# Autodesk Inventor assembly: sled
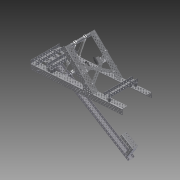
[picture p0: Inventor's stored thumbnail of the model, 180x180]
Saved by Autodesk Inventor 2014 SP1 (Build 180222100, 222)
## iProperties
Created: 2014-02-27
Part Number: sled
Document SubType Name: Assembly
Designer: Ryan
Author: Ryan
## Documents named in this file (28)
- C:\Users\Ryan\Desktop\sw\toss up 4th robot\intake\sled.iam
- C:\Users\Ryan\Desktop\sw\lib\Aperture VEX CAD Library\Metal\L Bar\2 x 35.ipt
- C:\Users\Ryan\Desktop\sw\lib\Aperture VEX CAD Library\Standoffs\BEAM-0500.ipt
- C:\Users\Ryan\Desktop\sw\lib\Aperture VEX CAD Library\Spacers\SPACER-0500-0125.ipt
- C:\Users\Ryan\Desktop\sw\lib\Aperture VEX CAD Library\Metal\C Channel\2 x 11.ipt
- C:\Users\Ryan\Desktop\sw\lib\Aperture VEX CAD Library\Metal\Plate\2 x 7.ipt
- C:\Users\Ryan\Desktop\sw\lib\Aperture VEX CAD Library\Metal\vex hinge\hinge.iam
- C:\Users\Ryan\Desktop\sw\lib\Aperture VEX CAD Library\Metal\C Channel\2 x 35.ipt
- C:\Users\Ryan\Desktop\sw\lib\Aperture VEX CAD Library\Spacers\SPACER-0500-0500.ipt
- C:\Users\Ryan\Desktop\sw\lib\Aperture VEX CAD Library\Metal\L Bar\2 x 14.ipt
- C:\Users\Ryan\Desktop\sw\lib\Aperture VEX CAD Library\Hardware\8-32\8-32_.375.ipt
- C:\Users\Ryan\Desktop\sw\lib\Aperture VEX CAD Library\Metal\Custom 1 bar\4 holes.ipt
- C:\Users\Ryan\Desktop\sw\lib\Aperture VEX CAD Library\Bearing Blocks\Bearing Block.ipt
- C:\Users\Ryan\Desktop\sw\lib\Aperture VEX CAD Library\Metal\Custom 1 bar\12.ipt
- C:\Users\Ryan\Desktop\sw\lib\Aperture VEX CAD Library\Pnuematics\Solenoid, Fwd, Reverse.iam
- C:\Users\Ryan\Desktop\sw\lib\Aperture VEX CAD Library\Shaft\5.5 inch shaft.ipt
- C:\Users\Ryan\Desktop\sw\lib\Aperture VEX CAD Library\Pnuematics\Cylinder, Bi-directional.iam
- C:\Users\Ryan\Desktop\sw\lib\Aperture VEX CAD Library\Pnuematics\End Gusset Fixed.ipt
- C:\Users\Ryan\Desktop\sw\lib\Aperture VEX CAD Library\Pnuematics\Cylinder, Bi-directional-Parts\Nut 8-32 Hex.ipt
- C:\Users\Ryan\Desktop\sw\lib\Aperture VEX CAD Library\Spacers\SPACER-0500-0250.ipt
- C:\Users\Ryan\Desktop\sw\lib\Aperture VEX CAD Library\Metal\Gussets\Lockbar.ipt
- C:\Users\Ryan\Desktop\sw\lib\Aperture VEX CAD Library\Spacers\SPACER-0500-0375.ipt
- C:\Users\Ryan\Desktop\sw\lib\Aperture VEX CAD Library\Standoffs\BEAM-1000.ipt
- C:\Users\Ryan\Desktop\sw\lib\Aperture VEX CAD Library\Metal\C Channel\2 x 5.ipt
- C:\Users\Ryan\Desktop\sw\lib\Aperture VEX CAD Library\Hardware\8-32\8-32 nylock.ipt
- C:\Users\Ryan\Desktop\sw\lib\Aperture VEX CAD Library\Hardware\8-32\8-32_.500.ipt
- C:\Users\Ryan\Desktop\sw\lib\Aperture VEX CAD Library\Hardware\6-32\6-32_.250.ipt
- C:\Users\Ryan\Desktop\sw\lib\Aperture VEX CAD Library\Hardware\6-32\thinner locknut.iam
## Components (158 placed, 26 different names)
1. 2 x 35:1 — Mate:1, Mate:2, Mate:3, Mate:6, Flush:1, Flush:2, Mate:29, Mate:30, Mate:31, Mate:32, Mate:33, Mate:34, Mate:133, Mate:217, Mate:219, Mate:244, Mate:247, Mate:266
2. BEAM-0500:1 — Mate:1, Mate:2, Mate:3, Mate:4, Mate:5
3. SPACER-0500-0125:1 — Mate:4, Mate:5, Mate:13, Mate:204, Mate:205, Mate:267
4. 2 x 11:1 — Mate:6, Flush:1, Flush:2, Mate:7, Flush:3, Flush:4, Mate:8, Flush:5, Flush:6, Mate:9, Flush:7, Flush:8, Mate:224, Mate:229
5. 2 x 7:1 — Mate:7, Flush:3, Flush:4, Mate:225, Mate:226, Mate:227
6. 2 x 35:2 — Mate:8, Flush:5, Flush:6, Mate:14, Mate:15, Mate:16, Mate:17, Mate:18, Mate:19, Mate:20, Mate:39, Mate:43, Mate:44, Mate:52, Mate:54, Flush:14, Mate:174, Mate:182, Mate:197, Mate:199, Mate:214, Mate:215, Mate:237, Mate:238, Mate:264
7. hinge:1 [sub-assembly] — Mate:9, Flush:7, Flush:8, Mate:10, Flush:9, Flush:10, Mate:94, Mate:95, Mate:96, Angle:2, Mate:136, Mate:137, Angle:4, Mate:158, Mate:162, Mate:163, Mate:192, Mate:220, Mate:221, Mate:222
8. 2 x 35:3 — Mate:10, Flush:9, Flush:10, Mate:80, Mate:81, Mate:82, Flush:12, Mate:129, Mate:159, Mate:160, Mate:183, Flush:15, Flush:16, Mate:269, Mate:271, Mate:277, Mate:279
9. BEAM-0500:2 — Mate:13, Mate:14
10. SPACER-0500-0125:2 — Mate:206, Mate:207, Mate:265
11. SPACER-0500-0500:1 — Mate:15, Mate:16, Mate:17, Mate:23, Mate:24, Mate:212
12. SPACER-0500-0500:2 — Mate:18, Mate:19, Mate:20, Mate:21, Mate:22, Mate:213, Mate:258
13. SPACER-0500-0125:3 — Mate:21, Mate:22, Mate:38
14. SPACER-0500-0125:4 — Mate:23, Mate:24, Mate:35, Mate:36, Mate:37
15. SPACER-0500-0500:3 — Mate:29, Mate:30, Mate:31, Mate:216
16. SPACER-0500-0500:4 — Mate:32, Mate:33, Mate:34, Mate:218
17. SPACER-0500-0125:5 — Mate:261
18. SPACER-0500-0125:6 — Mate:260
19. 2 x 11:2 — Mate:35, Mate:36, Mate:37, Mate:38, Mate:257, Mate:259, Mate:262, Mate:263
20. 2 x 14:1 — Mate:39, Mate:40, Mate:41, Mate:42, Mate:45, Mate:48, Mate:50, Mate:56, Mate:57, Mate:58, Mate:59, Mate:60, Mate:64, Mate:65, Mate:66, Mate:67, Mate:68, Angle:1, Flush:11, Mate:151, Mate:241, Mate:242, Mate:254, Mate:289, Mate:291, Mate:299
21. 8-32_.375:1 — Mate:40, Mate:41, Mate:42, Mate:43, Mate:44, Mate:134, Mate:239
22. 4 holes:1 — Mate:45, Mate:46, Mate:47, Mate:49, Mate:51, Mate:53, Mate:55
23. 8-32_.375:2 — Mate:46, Mate:47, Mate:48, Mate:49, Mate:50, Mate:255
24. 8-32_.375:3 — Mate:51, Mate:52, Mate:53, Mate:54, Mate:55, Mate:135, Mate:236
25. Bearing Block:1 — Mate:56, Mate:57, Mate:58, Mate:59, Mate:69, Mate:70, Mate:75, Mate:92, Mate:284, Mate:285, Mate:286, Mate:287, Mate:288, Mate:290
26. 12:1 — Mate:60, Mate:61, Mate:62, Mate:63, Mate:144, Mate:145, Mate:146
27. 8-32_.375:4 — Mate:61, Mate:62, Mate:63, Mate:64, Mate:65, Mate:240
28. Solenoid, Fwd, Reverse:1 [sub-assembly] — Mate:66, Mate:67, Mate:68, Angle:1, Angle:5, Mate:298, Mate:300
29. 5.5 inch shaft:1 — Flush:11, Mate:69, Mate:70
30. Cylinder, Bi-directional:1 [sub-assembly] — Mate:75, Mate:76, Mate:77, Mate:78, Mate:87, Mate:93, Mate:152
31. Nut 8-32 Hex:1 — Mate:185, Mate:186
32. End Gusset Fixed:2 — Mate:76, Mate:77, Mate:78, Mate:83, Mate:84, Mate:85, Mate:86, Mate:211
33. SPACER-0500-0125:7 — Mate:80, Mate:81, Mate:82, Mate:83, Mate:84, Mate:85, Mate:131, Mate:210
34. Nut 8-32 Hex:2 — Mate:86, Mate:87
35. SPACER-0500-0500:5 — Mate:88, Mate:89, Mate:90, Mate:153
36. SPACER-0500-0500:6 — Mate:89, Mate:91, Mate:92, Mate:93, Mate:132
37. SPACER-0500-0250:1 — Mate:88, Mate:90, Mate:91
38. Lockbar:1 — Mate:94, Mate:95, Mate:96, Angle:2, Mate:161, Mate:200, Mate:201, Flush:19
39. 2 x 14:2 — Mate:97, Mate:98, Mate:99, Mate:100, Mate:101, Mate:103, Mate:109, Mate:110, Mate:111, Mate:112, Mate:113, Angle:3, Mate:115, Mate:116, Mate:133, Mate:138, Mate:142, Mate:143, Mate:150, Mate:248, Mate:251, Mate:253, Mate:294, Mate:295, Mate:297
40. 8-32_.375:5 — Mate:97, Mate:98, Mate:99, Mate:134, Mate:246
41. 4 holes:2 — Mate:100, Mate:102, Mate:104, Mate:105, Mate:106, Mate:107, Mate:108
42. 8-32_.375:6 — Mate:101, Mate:102, Mate:103, Mate:104, Mate:105, Mate:250
43. 8-32_.375:7 — Mate:106, Mate:107, Mate:108, Mate:135, Mate:245
44. Bearing Block:2 — Mate:109, Mate:110, Mate:111, Mate:112, Mate:117, Mate:124, Mate:280, Mate:281, Mate:282, Mate:283, Mate:292, Mate:293
45. 12:2 — Mate:113, Mate:139, Mate:140, Mate:141, Mate:147, Mate:148, Mate:149
46. Solenoid, Fwd, Reverse:2 [sub-assembly] — Angle:3, Mate:115, Mate:116, Mate:138, Angle:5, Mate:296, Mate:302
47. Cylinder, Bi-directional:2 [sub-assembly] — Mate:117, Mate:118, Mate:119, Mate:120, Mate:123, Mate:132, Mate:154, Mate:185
48. End Gusset Fixed:3 — Mate:118, Mate:119, Mate:120, Flush:13, Mate:121, Mate:122, Mate:130, Mate:186, Mate:209
49. SPACER-0500-0125:8 — Flush:13, Mate:121, Mate:122, Mate:129, Mate:130, Mate:131, Mate:208
50. SPACER-0500-0500:7 — Mate:125, Mate:127, Mate:128, Mate:156
51. SPACER-0500-0500:8 — Mate:123, Mate:124, Mate:125, Mate:126
52. SPACER-0500-0250:2 — Mate:126, Mate:127, Mate:128
53. Lockbar:2 — Mate:136, Mate:137, Angle:4, Mate:164, Mate:189, Mate:192, Mate:193, Mate:202, Mate:203, Flush:19
54. 8-32_.375:8 — Mate:139, Mate:140, Mate:141, Mate:142, Mate:143, Mate:249
55. 8-32_.375:9 — Mate:144, Mate:145, Mate:146, Mate:150, Mate:252
56. 8-32_.375:10 — Mate:147, Mate:148, Mate:149, Mate:151, Mate:243
57. SPACER-0500-0500:9 — Mate:152, Mate:153, Mate:157
58. SPACER-0500-0375:1 — Mate:155, Mate:157
59. SPACER-0500-0500:10 — Mate:154, Mate:155, Mate:156
60. BEAM-1000:1 — Mate:158, Mate:159, Mate:160, Mate:166, Mate:168
61. BEAM-1000:2 — Mate:161, Mate:162, Mate:167, Mate:169
62. BEAM-1000:3 — Mate:163, Mate:164, Mate:165, Mate:170
63. SPACER-0500-0500:11 — Mate:165, Mate:170, Mate:230, Mate:231
64. SPACER-0500-0500:12 — Mate:166, Mate:168, Mate:232, Mate:233
65. SPACER-0500-0500:13 — Mate:167, Mate:169, Mate:234, Mate:235
66. 2 x 11:3 — Flush:14, Mate:173, Mate:175, Mate:176, Mate:179, Mate:180, Mate:181, Mate:274, Mate:275
67. 2 x 5:1 — Mate:183, Flush:15, Flush:16, Flush:17, Flush:18, Mate:184
68. 2 x 5:2 — Flush:17, Flush:18, Mate:184
69. 8-32_.375:22 — Mate:200, Mate:201, Mate:276
70. 8-32_.375:23 — Mate:202, Mate:203, Mate:278
71. 8-32_.375:24 — Mate:204, Mate:205
72. 8-32_.375:25 — Mate:206, Mate:207
73. 8-32_.375:26 — Mate:208, Mate:209, Mate:270
74. 8-32_.375:27 — Mate:210, Mate:211, Mate:268
75. 8-32_.375:28 — Mate:212, Mate:215, Mate:256
76. 8-32_.375:29 — Mate:213, Mate:214
77. 8-32_.375:30 — Mate:216, Mate:217
78. 8-32_.375:31 — Mate:218, Mate:219
79. 8-32_.375:37 — Mate:230, Mate:231
80. 8-32_.375:38 — Mate:232, Mate:233
81. 8-32_.375:39 — Mate:234, Mate:235
82. 8-32 nylock:8 — Mate:236, Mate:237
83. 8-32 nylock:9 — Mate:238, Mate:239
84. 8-32 nylock:10 — Mate:240, Mate:241
85. 8-32 nylock:11 — Mate:242, Mate:243
86. 8-32 nylock:12 — Mate:244, Mate:245
87. 8-32 nylock:13 — Mate:246, Mate:247
88. 8-32 nylock:14 — Mate:248, Mate:249
89. 8-32 nylock:15 — Mate:250, Mate:251
90. 8-32 nylock:16 — Mate:252, Mate:253
91. 8-32 nylock:17 — Mate:254, Mate:255
92. 8-32 nylock:18 — Mate:256, Mate:257
93. 8-32 nylock:19 — Mate:258, Mate:259
94. 8-32 nylock:20 — Mate:260, Mate:263
95. 8-32 nylock:21 — Mate:261, Mate:262
96. 8-32 nylock:22 — Mate:264, Mate:265
97. 8-32 nylock:23 — Mate:266, Mate:267
98. 8-32 nylock:24 — Mate:268, Mate:269
99. 8-32 nylock:25 — Mate:270, Mate:271
100. 8-32 nylock:34 — Mate:276, Mate:277
101. 8-32 nylock:35 — Mate:278, Mate:279
102. 8-32 nylock:36 — Mate:280, Mate:281
103. 8-32 nylock:37 — Mate:282, Mate:283
104. 8-32 nylock:38 — Mate:284, Mate:285
105. 8-32 nylock:39 — Mate:286, Mate:287
106. 8-32_.500:1 — Mate:288, Mate:289
107. 8-32_.500:2 — Mate:290, Mate:291
108. 8-32_.500:3 — Mate:293, Mate:295
109. 8-32_.500:4 — Mate:292, Mate:294
110. 6-32_.250:1 — Mate:296, Mate:297, Mate:303
111. 6-32_.250:2 — Mate:298, Mate:299, Mate:301
112. thinner locknut:1 [sub-assembly] — Mate:300, Mate:301
113. thinner locknut:2 [sub-assembly] — Mate:302, Mate:303
114. SPACER-0500-0500:15 — Mate:181, Mate:198, Mate:273
115. SPACER-0500-0125:10 — Mate:179, Mate:180
116. SPACER-0500-0125:9 — Mate:174, Mate:196
117. SPACER-0500-0500:14 — Mate:173, Mate:175, Mate:176, Mate:182, Mate:272
118. 8-32_.375:15 — Mate:198, Mate:199
119. 8-32_.375:14 — Mate:196, Mate:197
120. 8-32 nylock:27 — Mate:273, Mate:274
121. 8-32 nylock:26 — Mate:272, Mate:275
122. SPACER-0500-0500:16
123. SPACER-0500-0125:11
124. SPACER-0500-0125:12
125. SPACER-0500-0500:17
126. 8-32_.375:16
127. 8-32_.375:19
128. 8-32 nylock:28
129. 8-32 nylock:31
130. SPACER-0500-0500:18
131. SPACER-0500-0125:13
132. SPACER-0500-0125:14
133. SPACER-0500-0500:19
134. 8-32_.375:17
135. 8-32_.375:20
136. 8-32 nylock:29
137. 8-32 nylock:32
138. SPACER-0500-0500:20
139. SPACER-0500-0125:15
140. SPACER-0500-0125:16
141. SPACER-0500-0500:21
142. 8-32_.375:18
143. 8-32_.375:21
144. 8-32 nylock:30
145. 8-32 nylock:33
146. 8-32_.375:35 — Mate:225, Mate:226, Mate:227, Mate:228
147. 8-32 nylock:4 — Mate:228, Mate:229
148. 8-32_.375:36
149. 8-32 nylock:5
150. 8-32_.375:32 — Mate:220, Mate:221, Mate:222, Mate:223
151. 8-32_.375:12 — Mate:189, Mate:193
152. 8-32 nylock:1 — Mate:223, Mate:224
153. 8-32_.375:40
154. 8-32_.375:41
155. 8-32 nylock:6
156. 8-32_.375:42
157. 8-32_.375:43
158. 8-32 nylock:7
## Component patterns: (4 elements, first: SPACER-0500-0500:15 + SPACER-0500-0125:10 + SPACER-0500-0125:9 + SPACER-0500-0500:14 + 8-32_.375:15 + 8-32_.375:14 + 8-32 nylock:27 + 8-32 nylock:26), (2 elements, first: 8-32_.375:35 + 8-32 nylock:4), (3 elements, first: 8-32_.375:32 + 8-32_.375:12 + 8-32 nylock:1)
## Relationships (315: Mate 291, Flush 19, Angle 5)
- Mate:1: 2 x 35:1 ↔ BEAM-0500:1
- Mate:2 (2.3114 mm): 2 x 35:1 ↔ BEAM-0500:1
- Mate:3 (2.3114 mm): 2 x 35:1 ↔ BEAM-0500:1
- Mate:4: BEAM-0500:1 ↔ SPACER-0500-0125:1
- Mate:5: BEAM-0500:1 ↔ SPACER-0500-0125:1
- Mate:6: 2 x 35:1 ↔ 2 x 11:1
- Flush:1: 2 x 35:1 ↔ 2 x 11:1
- Flush:2: 2 x 35:1 ↔ 2 x 11:1
- Mate:7: 2 x 11:1 ↔ 2 x 7:1
- Flush:3: 2 x 11:1 ↔ 2 x 7:1
- Flush:4: 2 x 11:1 ↔ 2 x 7:1
- Mate:8: 2 x 11:1 ↔ 2 x 35:2
- Flush:5: 2 x 11:1 ↔ 2 x 35:2
- Flush:6: 2 x 11:1 ↔ 2 x 35:2
- Mate:9: 2 x 11:1 ↔ hinge:1
- Flush:7: 2 x 11:1 ↔ hinge:1
- Flush:8: 2 x 11:1 ↔ hinge:1
- Mate:10: hinge:1 ↔ 2 x 35:3
- Flush:9: hinge:1 ↔ 2 x 35:3
- Flush:10: hinge:1 ↔ 2 x 35:3
- [Mate]: BEAM-0500:2 ↔ SPACER-0500-0125:2
- [Mate]: BEAM-0500:2 ↔ SPACER-0500-0125:2
- Mate:13: SPACER-0500-0125:1 ↔ BEAM-0500:2
- Mate:14: 2 x 35:2 ↔ BEAM-0500:2
- Mate:15: 2 x 35:2 ↔ SPACER-0500-0500:1
- Mate:16 (2.3114 mm): 2 x 35:2 ↔ SPACER-0500-0500:1
- Mate:17 (2.3114 mm): 2 x 35:2 ↔ SPACER-0500-0500:1
- Mate:18 (2.3114 mm): 2 x 35:2 ↔ SPACER-0500-0500:2
- Mate:19 (2.3114 mm): 2 x 35:2 ↔ SPACER-0500-0500:2
- Mate:20: 2 x 35:2 ↔ SPACER-0500-0500:2
- Mate:21: SPACER-0500-0500:2 ↔ SPACER-0500-0125:3
- Mate:22: SPACER-0500-0500:2 ↔ SPACER-0500-0125:3
- Mate:23: SPACER-0500-0500:1 ↔ SPACER-0500-0125:4
- Mate:24: SPACER-0500-0500:1 ↔ SPACER-0500-0125:4
- [Mate]: SPACER-0500-0500:4 ↔ SPACER-0500-0125:5
- [Mate]: SPACER-0500-0500:4 ↔ SPACER-0500-0125:5
- [Mate]: SPACER-0500-0500:3 ↔ SPACER-0500-0125:6
- [Mate]: SPACER-0500-0500:3 ↔ SPACER-0500-0125:6
- Mate:29 (2.3114 mm): 2 x 35:1 ↔ SPACER-0500-0500:3
- Mate:30 (2.3114 mm): 2 x 35:1 ↔ SPACER-0500-0500:3
- Mate:31: 2 x 35:1 ↔ SPACER-0500-0500:3
- Mate:32: 2 x 35:1 ↔ SPACER-0500-0500:4
- Mate:33 (2.3114 mm): 2 x 35:1 ↔ SPACER-0500-0500:4
- Mate:34 (2.3114 mm): 2 x 35:1 ↔ SPACER-0500-0500:4
- Mate:35: SPACER-0500-0125:4 ↔ 2 x 11:2
- Mate:36 (2.3114 mm): SPACER-0500-0125:4 ↔ 2 x 11:2
- Mate:37 (2.3114 mm): SPACER-0500-0125:4 ↔ 2 x 11:2
- Mate:38 (2.3114 mm): SPACER-0500-0125:3 ↔ 2 x 11:2
- Mate:39: 2 x 35:2 ↔ 2 x 14:1
- Mate:40 (2.3114 mm): 2 x 14:1 ↔ 8-32_.375:1
- Mate:41 (2.3114 mm): 2 x 14:1 ↔ 8-32_.375:1
- Mate:42: 2 x 14:1 ↔ 8-32_.375:1
- Mate:43 (2.3114 mm): 2 x 35:2 ↔ 8-32_.375:1
- Mate:44 (2.3114 mm): 2 x 35:2 ↔ 8-32_.375:1
- Mate:45: 2 x 14:1 ↔ 4 holes:1
- Mate:46 (2.3114 mm): 4 holes:1 ↔ 8-32_.375:2
- Mate:47 (2.3114 mm): 4 holes:1 ↔ 8-32_.375:2
- Mate:48 (2.3114 mm): 2 x 14:1 ↔ 8-32_.375:2
- Mate:49: 4 holes:1 ↔ 8-32_.375:2
- Mate:50 (2.3114 mm): 2 x 14:1 ↔ 8-32_.375:2
- Mate:51 (2.3114 mm): 4 holes:1 ↔ 8-32_.375:3
- Mate:52 (2.3114 mm): 2 x 35:2 ↔ 8-32_.375:3
- Mate:53 (2.3114 mm): 4 holes:1 ↔ 8-32_.375:3
- Mate:54 (2.3114 mm): 2 x 35:2 ↔ 8-32_.375:3
- Mate:55: 4 holes:1 ↔ 8-32_.375:3
- Mate:56: 2 x 14:1 ↔ Bearing Block:1
- Mate:57 (2.3114 mm): 2 x 14:1 ↔ Bearing Block:1
- Mate:58 (2.3114 mm): 2 x 14:1 ↔ Bearing Block:1
- Mate:59 (2.3114 mm): 2 x 14:1 ↔ Bearing Block:1
- Mate:60: 2 x 14:1 ↔ 12:1
- Mate:61 (2.3114 mm): 12:1 ↔ 8-32_.375:4
- Mate:62 (2.3114 mm): 12:1 ↔ 8-32_.375:4
- Mate:63: 12:1 ↔ 8-32_.375:4
- Mate:64 (2.3114 mm): 2 x 14:1 ↔ 8-32_.375:4
- Mate:65 (2.3114 mm): 2 x 14:1 ↔ 8-32_.375:4
- Mate:66: 2 x 14:1 ↔ Solenoid, Fwd, Reverse:1
- Mate:67 (2.3114 mm): 2 x 14:1 ↔ Solenoid, Fwd, Reverse:1
- Mate:68 (2.3114 mm): 2 x 14:1 ↔ Solenoid, Fwd, Reverse:1
- Angle:1 (0 deg): 2 x 14:1 ↔ Solenoid, Fwd, Reverse:1
- Flush:11: 2 x 14:1 ↔ 5.5 inch shaft:1
- Mate:69 (-1.5875 mm): Bearing Block:1 ↔ 5.5 inch shaft:1
- Mate:70 (-1.5875 mm): Bearing Block:1 ↔ 5.5 inch shaft:1
- Mate:75: Bearing Block:1 ↔ Cylinder, Bi-directional:1
- Mate:76: Cylinder, Bi-directional:1 ↔ End Gusset Fixed:2
- Mate:77 (2.3114 mm): Cylinder, Bi-directional:1 ↔ End Gusset Fixed:2
- Mate:78 (2.3114 mm): Cylinder, Bi-directional:1 ↔ End Gusset Fixed:2
- Mate:80: 2 x 35:3 ↔ SPACER-0500-0125:7
- Mate:81 (2.3114 mm): 2 x 35:3 ↔ SPACER-0500-0125:7
- Mate:82 (2.3114 mm): 2 x 35:3 ↔ SPACER-0500-0125:7
- Mate:83 (2.3114 mm): End Gusset Fixed:2 ↔ SPACER-0500-0125:7
- Mate:84 (2.3114 mm): End Gusset Fixed:2 ↔ SPACER-0500-0125:7
- Mate:85: End Gusset Fixed:2 ↔ SPACER-0500-0125:7
- Mate:86: End Gusset Fixed:2 ↔ Nut 8-32 Hex:2
- Mate:87: Cylinder, Bi-directional:1 ↔ Nut 8-32 Hex:2
- Mate:88: SPACER-0500-0500:5 ↔ SPACER-0500-0250:1
- Mate:89: SPACER-0500-0500:5 ↔ SPACER-0500-0500:6
- Mate:90: SPACER-0500-0500:5 ↔ SPACER-0500-0250:1
- Mate:91: SPACER-0500-0500:6 ↔ SPACER-0500-0250:1
- Mate:92: Bearing Block:1 ↔ SPACER-0500-0500:6
- Mate:93: Cylinder, Bi-directional:1 ↔ SPACER-0500-0500:6
- Mate:94: hinge:1 ↔ Lockbar:1
- Mate:95 (2.3114 mm): hinge:1 ↔ Lockbar:1
- Mate:96 (2.3114 mm): hinge:1 ↔ Lockbar:1
- Angle:2 (45 deg): hinge:1 ↔ Lockbar:1
- Flush:12 (-12.7 mm): 2 x 35:3
- Mate:97: 2 x 14:2 ↔ 8-32_.375:5
- Mate:98 (2.3114 mm): 2 x 14:2 ↔ 8-32_.375:5
- Mate:99 (2.3114 mm): 2 x 14:2 ↔ 8-32_.375:5
- Mate:100: 2 x 14:2 ↔ 4 holes:2
- Mate:101 (2.3114 mm): 2 x 14:2 ↔ 8-32_.375:6
- Mate:102: 4 holes:2 ↔ 8-32_.375:6
- Mate:103 (2.3114 mm): 2 x 14:2 ↔ 8-32_.375:6
- Mate:104 (2.3114 mm): 4 holes:2 ↔ 8-32_.375:6
- Mate:105 (2.3114 mm): 4 holes:2 ↔ 8-32_.375:6
- Mate:106: 4 holes:2 ↔ 8-32_.375:7
- Mate:107 (2.3114 mm): 4 holes:2 ↔ 8-32_.375:7
- Mate:108 (2.3114 mm): 4 holes:2 ↔ 8-32_.375:7
- Mate:109 (2.3114 mm): 2 x 14:2 ↔ Bearing Block:2
- Mate:110 (2.3114 mm): 2 x 14:2 ↔ Bearing Block:2
- Mate:111 (2.3114 mm): 2 x 14:2 ↔ Bearing Block:2
- Mate:112: 2 x 14:2 ↔ Bearing Block:2
- Mate:113: 2 x 14:2 ↔ 12:2
- Angle:3 (0 deg): 2 x 14:2 ↔ Solenoid, Fwd, Reverse:2
- Mate:115 (2.3114 mm): 2 x 14:2 ↔ Solenoid, Fwd, Reverse:2
- Mate:116: 2 x 14:2 ↔ Solenoid, Fwd, Reverse:2
- Mate:117: Bearing Block:2 ↔ Cylinder, Bi-directional:2
- Mate:118 (2.3114 mm): Cylinder, Bi-directional:2 ↔ End Gusset Fixed:3
- Mate:119 (2.3114 mm): Cylinder, Bi-directional:2 ↔ End Gusset Fixed:3
- Mate:120: Cylinder, Bi-directional:2 ↔ End Gusset Fixed:3
- Flush:13: End Gusset Fixed:3 ↔ SPACER-0500-0125:8
- Mate:121 (2.3114 mm): End Gusset Fixed:3 ↔ SPACER-0500-0125:8
- Mate:122 (2.3114 mm): End Gusset Fixed:3 ↔ SPACER-0500-0125:8
- Mate:123: Cylinder, Bi-directional:2 ↔ SPACER-0500-0500:8
- Mate:124: Bearing Block:2 ↔ SPACER-0500-0500:8
- Mate:125: SPACER-0500-0500:7 ↔ SPACER-0500-0500:8
- Mate:126: SPACER-0500-0500:8 ↔ SPACER-0500-0250:2
- Mate:127: SPACER-0500-0500:7 ↔ SPACER-0500-0250:2
- Mate:128: SPACER-0500-0500:7 ↔ SPACER-0500-0250:2
- Mate:129: 2 x 35:3 ↔ SPACER-0500-0125:8
- Mate:130: End Gusset Fixed:3 ↔ SPACER-0500-0125:8
- Mate:131: SPACER-0500-0125:7 ↔ SPACER-0500-0125:8
- Mate:132: SPACER-0500-0500:6 ↔ Cylinder, Bi-directional:2
- Mate:133: 2 x 35:1 ↔ 2 x 14:2
- Mate:134: 8-32_.375:1 ↔ 8-32_.375:5
- Mate:135: 8-32_.375:3 ↔ 8-32_.375:7
- Mate:136 (2.3114 mm): hinge:1 ↔ Lockbar:2
- Mate:137 (2.3114 mm): hinge:1 ↔ Lockbar:2
- Angle:4 (-45 deg): hinge:1 ↔ Lockbar:2
- Mate:138 (2.3114 mm): 2 x 14:2 ↔ Solenoid, Fwd, Reverse:2
- Angle:5 (0 deg): Solenoid, Fwd, Reverse:1 ↔ Solenoid, Fwd, Reverse:2
- Mate:139 (2.3114 mm): 12:2 ↔ 8-32_.375:8
- Mate:140 (2.3114 mm): 12:2 ↔ 8-32_.375:8
- Mate:141: 12:2 ↔ 8-32_.375:8
- Mate:142 (2.3114 mm): 2 x 14:2 ↔ 8-32_.375:8
- Mate:143 (2.3114 mm): 2 x 14:2 ↔ 8-32_.375:8
- Mate:144 (2.3114 mm): 12:1 ↔ 8-32_.375:9
- Mate:145 (2.3114 mm): 12:1 ↔ 8-32_.375:9
- Mate:146: 12:1 ↔ 8-32_.375:9
- Mate:147 (2.3114 mm): 12:2 ↔ 8-32_.375:10
- Mate:148 (2.3114 mm): 12:2 ↔ 8-32_.375:10
- Mate:149: 12:2 ↔ 8-32_.375:10
- Mate:150 (2.3114 mm): 2 x 14:2 ↔ 8-32_.375:9
- Mate:151 (2.3114 mm): 2 x 14:1 ↔ 8-32_.375:10
- Mate:152: Cylinder, Bi-directional:1 ↔ SPACER-0500-0500:9
- Mate:153: SPACER-0500-0500:5 ↔ SPACER-0500-0500:9
- Mate:154: Cylinder, Bi-directional:2 ↔ SPACER-0500-0500:10
- Mate:155: SPACER-0500-0375:1 ↔ SPACER-0500-0500:10
- Mate:156: SPACER-0500-0500:7 ↔ SPACER-0500-0500:10
- Mate:157 (0.6223 mm): SPACER-0500-0500:9 ↔ SPACER-0500-0375:1
- Mate:158 (2.3114 mm): hinge:1 ↔ BEAM-1000:1
- Mate:159: 2 x 35:3 ↔ BEAM-1000:1
- Mate:160 (2.3114 mm): 2 x 35:3 ↔ BEAM-1000:1
- Mate:161: Lockbar:1 ↔ BEAM-1000:2
- Mate:162: hinge:1 ↔ BEAM-1000:2
- Mate:163: hinge:1 ↔ BEAM-1000:3
- Mate:164: Lockbar:2 ↔ BEAM-1000:3
- Mate:165: BEAM-1000:3 ↔ SPACER-0500-0500:11
- Mate:166: BEAM-1000:1 ↔ SPACER-0500-0500:12
- Mate:167: BEAM-1000:2 ↔ SPACER-0500-0500:13
- Mate:168: BEAM-1000:1 ↔ SPACER-0500-0500:12
- Mate:169: BEAM-1000:2 ↔ SPACER-0500-0500:13
- Mate:170: BEAM-1000:3 ↔ SPACER-0500-0500:11
- Flush:14: 2 x 35:2 ↔ 2 x 11:3
- [Mate]: SPACER-0500-0125:9 ↔ SPACER-0500-0500:14
- [Mate]: SPACER-0500-0125:9 ↔ SPACER-0500-0500:14
- Mate:173: 2 x 11:3 ↔ SPACER-0500-0500:14
- Mate:174: 2 x 35:2 ↔ SPACER-0500-0125:9
- Mate:175 (2.3114 mm): 2 x 11:3 ↔ SPACER-0500-0500:14
- Mate:176 (2.3114 mm): 2 x 11:3 ↔ SPACER-0500-0500:14
- [Mate]: SPACER-0500-0500:15 ↔ SPACER-0500-0125:10
- [Mate]: SPACER-0500-0500:15 ↔ SPACER-0500-0125:10
- Mate:179 (2.3114 mm): 2 x 11:3 ↔ SPACER-0500-0125:10
- Mate:180: 2 x 11:3 ↔ SPACER-0500-0125:10
- Mate:181 (2.3114 mm): 2 x 11:3 ↔ SPACER-0500-0500:15
- Mate:182 (2.3114 mm): 2 x 35:2 ↔ SPACER-0500-0500:14
- Mate:183: 2 x 35:3 ↔ 2 x 5:1
- Flush:15: 2 x 35:3 ↔ 2 x 5:1
- Flush:16: 2 x 35:3 ↔ 2 x 5:1
- Flush:17: 2 x 5:1 ↔ 2 x 5:2
- Flush:18: 2 x 5:1 ↔ 2 x 5:2
- Mate:184: 2 x 5:1 ↔ 2 x 5:2
- Mate:185: Nut 8-32 Hex:1 ↔ Cylinder, Bi-directional:2
- Mate:186: Nut 8-32 Hex:1 ↔ End Gusset Fixed:3
- Mate:189: Lockbar:2 ↔ 8-32_.375:12
- Mate:192: hinge:1 ↔ Lockbar:2
- Mate:193: Lockbar:2 ↔ 8-32_.375:12
- Mate:196: SPACER-0500-0125:9 ↔ 8-32_.375:14
- Mate:197: 2 x 35:2 ↔ 8-32_.375:14
- Mate:198: SPACER-0500-0500:15 ↔ 8-32_.375:15
- Mate:199: 2 x 35:2 ↔ 8-32_.375:15
- Mate:200: Lockbar:1 ↔ 8-32_.375:22
- Mate:201: Lockbar:1 ↔ 8-32_.375:22
- Mate:202: Lockbar:2 ↔ 8-32_.375:23
- Mate:203: Lockbar:2 ↔ 8-32_.375:23
- Mate:204: SPACER-0500-0125:1 ↔ 8-32_.375:24
- Mate:205: SPACER-0500-0125:1 ↔ 8-32_.375:24
- Mate:206: SPACER-0500-0125:2 ↔ 8-32_.375:25
- Mate:207: SPACER-0500-0125:2 ↔ 8-32_.375:25
- Mate:208: SPACER-0500-0125:8 ↔ 8-32_.375:26
- Mate:209: End Gusset Fixed:3 ↔ 8-32_.375:26
- Mate:210: SPACER-0500-0125:7 ↔ 8-32_.375:27
- Mate:211: End Gusset Fixed:2 ↔ 8-32_.375:27
- Mate:212: SPACER-0500-0500:1 ↔ 8-32_.375:28
- Mate:213: SPACER-0500-0500:2 ↔ 8-32_.375:29
- Mate:214: 2 x 35:2 ↔ 8-32_.375:29
- Mate:215: 2 x 35:2 ↔ 8-32_.375:28
- Mate:216: SPACER-0500-0500:3 ↔ 8-32_.375:30
- Mate:217: 2 x 35:1 ↔ 8-32_.375:30
- Mate:218: SPACER-0500-0500:4 ↔ 8-32_.375:31
- Mate:219: 2 x 35:1 ↔ 8-32_.375:31
- Mate:220 (2.3114 mm): hinge:1 ↔ 8-32_.375:32
- Mate:221 (2.3114 mm): hinge:1 ↔ 8-32_.375:32
- Mate:222: hinge:1 ↔ 8-32_.375:32
- Mate:223: 8-32_.375:32 ↔ 8-32 nylock:1
- Mate:224: 2 x 11:1 ↔ 8-32 nylock:1
- Mate:225 (2.3114 mm): 2 x 7:1 ↔ 8-32_.375:35
- Mate:226 (2.3114 mm): 2 x 7:1 ↔ 8-32_.375:35
- Mate:227: 2 x 7:1 ↔ 8-32_.375:35
- Mate:228: 8-32_.375:35 ↔ 8-32 nylock:4
- Mate:229: 2 x 11:1 ↔ 8-32 nylock:4
- Mate:230: SPACER-0500-0500:11 ↔ 8-32_.375:37
- Mate:231: SPACER-0500-0500:11 ↔ 8-32_.375:37
- Mate:232: SPACER-0500-0500:12 ↔ 8-32_.375:38
- Mate:233: SPACER-0500-0500:12 ↔ 8-32_.375:38
- Mate:234: SPACER-0500-0500:13 ↔ 8-32_.375:39
- Mate:235: SPACER-0500-0500:13 ↔ 8-32_.375:39
- Flush:19: Lockbar:1 ↔ Lockbar:2
- Mate:236: 8-32_.375:3 ↔ 8-32 nylock:8
- Mate:237: 2 x 35:2 ↔ 8-32 nylock:8
- Mate:238: 2 x 35:2 ↔ 8-32 nylock:9
- Mate:239: 8-32_.375:1 ↔ 8-32 nylock:9
- Mate:240: 8-32_.375:4 ↔ 8-32 nylock:10
- Mate:241: 2 x 14:1 ↔ 8-32 nylock:10
- Mate:242: 2 x 14:1 ↔ 8-32 nylock:11
- Mate:243: 8-32_.375:10 ↔ 8-32 nylock:11
- Mate:244: 2 x 35:1 ↔ 8-32 nylock:12
- Mate:245: 8-32_.375:7 ↔ 8-32 nylock:12
- Mate:246: 8-32_.375:5 ↔ 8-32 nylock:13
- Mate:247: 2 x 35:1 ↔ 8-32 nylock:13
- Mate:248: 2 x 14:2 ↔ 8-32 nylock:14
- Mate:249: 8-32_.375:8 ↔ 8-32 nylock:14
- Mate:250: 8-32_.375:6 ↔ 8-32 nylock:15
- Mate:251: 2 x 14:2 ↔ 8-32 nylock:15
- Mate:252: 8-32_.375:9 ↔ 8-32 nylock:16
- Mate:253: 2 x 14:2 ↔ 8-32 nylock:16
- Mate:254: 2 x 14:1 ↔ 8-32 nylock:17
- Mate:255: 8-32_.375:2 ↔ 8-32 nylock:17
- Mate:256: 8-32_.375:28 ↔ 8-32 nylock:18
- Mate:257: 2 x 11:2 ↔ 8-32 nylock:18
- Mate:258: SPACER-0500-0500:2 ↔ 8-32 nylock:19
- Mate:259: 2 x 11:2 ↔ 8-32 nylock:19
- Mate:260: SPACER-0500-0125:6 ↔ 8-32 nylock:20
- Mate:261: SPACER-0500-0125:5 ↔ 8-32 nylock:21
- Mate:262: 2 x 11:2 ↔ 8-32 nylock:21
- Mate:263: 2 x 11:2 ↔ 8-32 nylock:20
- Mate:264: 2 x 35:2 ↔ 8-32 nylock:22
- Mate:265: SPACER-0500-0125:2 ↔ 8-32 nylock:22
- Mate:266: 2 x 35:1 ↔ 8-32 nylock:23
- Mate:267: SPACER-0500-0125:1 ↔ 8-32 nylock:23
- Mate:268: 8-32_.375:27 ↔ 8-32 nylock:24
- Mate:269: 2 x 35:3 ↔ 8-32 nylock:24
- Mate:270: 8-32_.375:26 ↔ 8-32 nylock:25
- Mate:271: 2 x 35:3 ↔ 8-32 nylock:25
- Mate:272: SPACER-0500-0500:14 ↔ 8-32 nylock:26
- Mate:273: SPACER-0500-0500:15 ↔ 8-32 nylock:27
- Mate:274: 2 x 11:3 ↔ 8-32 nylock:27
- Mate:275: 2 x 11:3 ↔ 8-32 nylock:26
- Mate:276: 8-32_.375:22 ↔ 8-32 nylock:34
- Mate:277: 2 x 35:3 ↔ 8-32 nylock:34
- Mate:278: 8-32_.375:23 ↔ 8-32 nylock:35
- Mate:279: 2 x 35:3 ↔ 8-32 nylock:35
- Mate:280: Bearing Block:2 ↔ 8-32 nylock:36
- Mate:281: Bearing Block:2 ↔ 8-32 nylock:36
- Mate:282: Bearing Block:2 ↔ 8-32 nylock:37
- Mate:283: Bearing Block:2 ↔ 8-32 nylock:37
- Mate:284: Bearing Block:1 ↔ 8-32 nylock:38
- Mate:285: Bearing Block:1 ↔ 8-32 nylock:38
- Mate:286: Bearing Block:1 ↔ 8-32 nylock:39
- Mate:287: Bearing Block:1 ↔ 8-32 nylock:39
- Mate:288: Bearing Block:1 ↔ 8-32_.500:1
- Mate:289: 2 x 14:1 ↔ 8-32_.500:1
- Mate:290: Bearing Block:1 ↔ 8-32_.500:2
- Mate:291: 2 x 14:1 ↔ 8-32_.500:2
- Mate:292: Bearing Block:2 ↔ 8-32_.500:4
- Mate:293: Bearing Block:2 ↔ 8-32_.500:3
- Mate:294: 2 x 14:2 ↔ 8-32_.500:4
- Mate:295: 2 x 14:2 ↔ 8-32_.500:3
- Mate:296: Solenoid, Fwd, Reverse:2 ↔ 6-32_.250:1
- Mate:297: 2 x 14:2 ↔ 6-32_.250:1
- Mate:298: Solenoid, Fwd, Reverse:1 ↔ 6-32_.250:2
- Mate:299: 2 x 14:1 ↔ 6-32_.250:2
- Mate:300: Solenoid, Fwd, Reverse:1 ↔ thinner locknut:1
- Mate:301: 6-32_.250:2 ↔ thinner locknut:1
- Mate:302: Solenoid, Fwd, Reverse:2 ↔ thinner locknut:2
- Mate:303: 6-32_.250:1 ↔ thinner locknut:2
## Named parameters: q = 2.3114 mm, d20_d3 = 0 mm, d21_d4 = 0 mm, d34_d30 = 0 mm, d35_d31 = 0 mm, d36_d32 = 0 mm, d37_d33 = 0 mm, d195_d30 = 0 mm, d196_d31 = 0 mm, d201_d195_d30 = 0 mm, d202_d196_d31 = 0 mm
